# Autodesk Inventor assembly: KPA4CUNPL
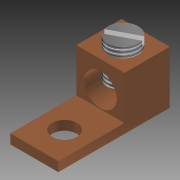
[picture p0: Inventor's stored thumbnail of the model, 180x180]
Saved by Autodesk Inventor 2013 (Build 170138000, 138)
## iProperties
Shininess: 64.0
Angle Display Precision: 2
Document Length Units: 11272
Document Angle Units: 11279
Document Time Units: 11290
Document Mass Units: 11286
Document Length Units Precision: 3
Document Angle Units Precision: 2
Category: Electrical
Company: Autodesk Inc.
Created: 2012-12-07
Part Number: KPA4CUNPL
Catalog Web Link: http://www.burndy.com/site-search.aspx?cx=002899303449139187703%3Ae9jb50hrnuc&cof=FORID%3A10&ie=UTF-8&q=kpa4cunpl&SearchType=PartNumber&go.x=36&go.y=12
Description: Terminal lug, 6-14ga solderless lug, mechanical
Vendor: FCI Burndy
Document SubType Name: Assembly
Designer: Autodesk Inc.
Density: 0.0
Volumn: 0.0
Area: 0.0
PropertySet Name: Model Information
Control State: 0
Master: False
Checked Out: False
Author: Autodesk Inc.
## Documents named in this file (3)
- C:\Data Folder\FIRST 2013\FIRST KOP\Parts\Electrical\ELEC_Terminal Lug _KPA4CUNPL.iam
- C:\Data Folder\FIRST 2013\FIRST KOP\Parts\Electrical\Terminal Battery.ipt
- C:\Data Folder\FIRST 2013\FIRST KOP\Parts\Electrical\Terminal Screw.ipt
## Components (2 placed, 2 different names)
1. Terminal Battery:1 — Mate:1, Flush:1
2. Terminal Screw:1 — Mate:1, Flush:1
## Relationships (2: Mate 1, Flush 1)
- Mate:1: Terminal Battery:1 ↔ Terminal Screw:1
- Flush:1 (-2.54 mm): Terminal Battery:1 ↔ Terminal Screw:1
